# Autodesk Inventor assembly: Frezowanie No.1
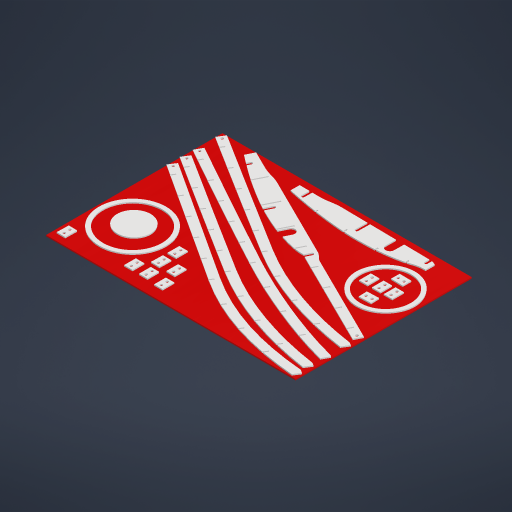
[picture p0: Inventor's stored thumbnail of the model, 512x512]
Saved by Autodesk Inventor 2023 (Build 270158000, 158)
## iProperties
Created: 2023-04-06
Part Number: Frezowanie No.1
Document SubType Name: Assembly
Designer: szykr
Author: szykr
## Documents named in this file (23)
- D:\Folder Instalacyjny\GitHub Pliki\Solaris\new model\Frez\Frezowanie No.1.iam
- D:\Folder Instalacyjny\GitHub Pliki\Solaris\new model\Frez\Laminat297x210.ipt
- D:\Folder Instalacyjny\GitHub Pliki\Solaris\new model\Frez\Dlugie party(32-47)\Solid32.ipt
- D:\Folder Instalacyjny\GitHub Pliki\Solaris\new model\Frez\Dlugie party(32-47)\Solid34.ipt
- D:\Folder Instalacyjny\GitHub Pliki\Solaris\new model\Frez\Dlugie party(32-47)\Solid36.ipt
- D:\Folder Instalacyjny\GitHub Pliki\Solaris\new model\Frez\Dlugie party(32-47)\Solid38.ipt
- D:\Folder Instalacyjny\GitHub Pliki\Solaris\new model\Frez\Dlugie party(32-47)\Solid42.ipt
- D:\Folder Instalacyjny\GitHub Pliki\Solaris\new model\Frez\Troche Mniejsze(2-31)\Solid2.ipt
- D:\Folder Instalacyjny\GitHub Pliki\Solaris\new model\Frez\Troche Mniejsze(2-31)\Solid3.ipt
- D:\Folder Instalacyjny\GitHub Pliki\Solaris\new model\Frez\Troche Mniejsze(2-31)\Solid4.ipt
- D:\Folder Instalacyjny\GitHub Pliki\Solaris\new model\Frez\Troche Mniejsze(2-31)\Solid28.ipt
- D:\Folder Instalacyjny\GitHub Pliki\Solaris\new model\Frez\Kuplungi(48-65)\Solid48.ipt
- D:\Folder Instalacyjny\GitHub Pliki\Solaris\new model\Frez\Kuplungi(48-65)\Solid49.ipt
- D:\Folder Instalacyjny\GitHub Pliki\Solaris\new model\Frez\Kuplungi(48-65)\Solid50.ipt
- D:\Folder Instalacyjny\GitHub Pliki\Solaris\new model\Frez\Kuplungi(48-65)\Solid51.ipt
- D:\Folder Instalacyjny\GitHub Pliki\Solaris\new model\Frez\Kuplungi(48-65)\Solid52.ipt
- D:\Folder Instalacyjny\GitHub Pliki\Solaris\new model\Frez\Kuplungi(48-65)\Solid53.ipt
- D:\Folder Instalacyjny\GitHub Pliki\Solaris\new model\Frez\Kuplungi(48-65)\Solid54.ipt
- D:\Folder Instalacyjny\GitHub Pliki\Solaris\new model\Frez\Kuplungi(48-65)\Solid55.ipt
- D:\Folder Instalacyjny\GitHub Pliki\Solaris\new model\Frez\Kuplungi(48-65)\Solid56.ipt
- D:\Folder Instalacyjny\GitHub Pliki\Solaris\new model\Frez\Kuplungi(48-65)\Solid57.ipt
- D:\Folder Instalacyjny\GitHub Pliki\Solaris\new model\Frez\Kuplungi(48-65)\Solid60.ipt
- D:\Folder Instalacyjny\GitHub Pliki\Solaris\new model\Frez\Kuplungi(48-65)\Solid61.ipt
## Components (22 placed, 22 different names)
1. Laminat297x210:1 — Angle:1, Mate:1, Angle:3, Mate:2, Angle:5, Mate:3, Angle:6, Mate:4, Mate:5, Mate:6, Mate:7, Mate:8, Mate:9, Mate:10, Mate:11, Mate:12, Mate:13, Mate:14, Mate:15, Mate:16, Mate:17, Mate:18, Mate:19, Mate:20, Mate:21
2. Solid32:1 — Angle:1, Mate:1
3. Solid34:1 — Angle:3, Mate:2
4. Solid36:1 — Angle:5, Mate:3
5. Solid38:1 — Angle:6, Mate:4
6. Solid42:1 — Mate:5
7. Solid2:1 — Mate:6
8. Solid3:1 — Mate:7
9. Solid4:1 — Mate:8
10. Solid28:1 — Mate:9
11. Solid48:1 — Mate:10
12. Solid49:1 — Mate:11
13. Solid50:1 — Mate:12
14. Solid51:1 — Mate:13
15. Solid52:1 — Mate:14
16. Solid53:1 — Mate:15
17. Solid54:1 — Mate:16
18. Solid55:1 — Mate:17
19. Solid56:1 — Mate:18
20. Solid57:1 — Mate:19
21. Solid60:1 — Mate:20
22. Solid61:1 — Mate:21
## Relationships (25: Mate 21, Angle 4)
- Angle:1 (180 deg): Laminat297x210:1 ↔ Solid32:1
- Mate:1: Laminat297x210:1 ↔ Solid32:1
- Angle:3 (180 deg): Laminat297x210:1 ↔ Solid34:1
- Mate:2: Laminat297x210:1 ↔ Solid34:1
- Angle:5 (0 deg): Laminat297x210:1 ↔ Solid36:1
- Mate:3: Laminat297x210:1 ↔ Solid36:1
- Angle:6 (0 deg): Laminat297x210:1 ↔ Solid38:1
- Mate:4: Laminat297x210:1 ↔ Solid38:1
- Mate:5: Laminat297x210:1 ↔ Solid42:1
- Mate:6: Laminat297x210:1 ↔ Solid2:1
- Mate:7: Laminat297x210:1 ↔ Solid3:1
- Mate:8: Laminat297x210:1 ↔ Solid4:1
- Mate:9: Laminat297x210:1 ↔ Solid28:1
- Mate:10: Laminat297x210:1 ↔ Solid48:1
- Mate:11: Laminat297x210:1 ↔ Solid49:1
- Mate:12: Laminat297x210:1 ↔ Solid50:1
- Mate:13: Laminat297x210:1 ↔ Solid51:1
- Mate:14: Laminat297x210:1 ↔ Solid52:1
- Mate:15: Laminat297x210:1 ↔ Solid53:1
- Mate:16: Laminat297x210:1 ↔ Solid54:1
- Mate:17: Laminat297x210:1 ↔ Solid55:1
- Mate:18: Laminat297x210:1 ↔ Solid56:1
- Mate:19: Laminat297x210:1 ↔ Solid57:1
- Mate:20: Laminat297x210:1 ↔ Solid60:1
- Mate:21: Laminat297x210:1 ↔ Solid61:1
